# Autodesk Inventor assembly: saddle cart
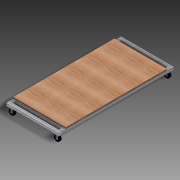
[picture p0: Inventor's stored thumbnail of the model, 180x180]
Saved by Autodesk Inventor 2013 (Build 170138000, 138)
## iProperties
Created: 2013-01-03
Part Number: saddle cart
Document SubType Name: Assembly
Designer: Arpan
Author: Arpan
## Documents named in this file (7)
- C:\Users\Arpan\Documents\Robotics 2013\Cart- Take 2\saddle cart.iam
- C:\Users\Arpan\Documents\Robotics 2013\Cart- Take 2\56 piece.ipt
- C:\Users\Arpan\Documents\Robotics 2013\Cart- Take 2\28 piece.ipt
- C:\Users\Arpan\Documents\Robotics 2013\Cart- Take 2\25 piece.ipt
- C:\Users\Arpan\Documents\Robotics 2013\Cart- Take 2\2.5 piece.ipt
- C:\Users\Arpan\Documents\Robotics 2013\Cart- Take 2\saddle cart top.ipt
- C:\Users\Arpan\Documents\Robotics 2013\Cart- Take 2\small caster\small caster.iam
## Components (15 placed, 6 different names)
1. 56 piece:1 — Mate:1, Flush:1, Flush:2, Mate:4, Flush:7, Mate:5, Flush:8, Mate:14, Mate:15, Flush:14, Flush:18, Flush:22
2. 56 piece:2 — Flush:3, Flush:4, Mate:2, Mate:3, Flush:5, Flush:6, Mate:12, Mate:13, Flush:15, Mate:19, Flush:20
3. 28 piece:1 — Mate:1, Flush:1, Flush:2, Flush:3, Flush:4, Mate:2, Mate:17, Flush:16, Mate:18, Flush:17
4. 28 piece:2 — Mate:3, Flush:5, Flush:6, Mate:7, Flush:19, Mate:20, Flush:21
5. 25 piece:1 — Mate:4, Flush:7, Mate:6, Mate:7, Flush:11, Mate:10, Flush:12, Mate:11, Mate:16
6. 25 piece:2 — Mate:5, Flush:8, Mate:6, Mate:8, Flush:9, Flush:10, Mate:9, Flush:13
7. 2.5 piece:1 — Mate:8, Flush:9, Mate:13
8. 2.5 piece:2 — Flush:10, Mate:9, Mate:14
9. 2.5 piece:3 — Flush:11, Mate:10, Mate:15
10. 2.5 piece:4 — Flush:12, Mate:11, Mate:12
11. saddle cart top:1 — Mate:16, Flush:13, Flush:14
12. small caster:1 [sub-assembly] — Mate:19, Flush:19, Flush:20
13. small caster:2 [sub-assembly] — Mate:17, Flush:15, Flush:16
14. small caster:3 [sub-assembly] — Mate:18, Flush:17, Flush:18
15. small caster:4 [sub-assembly] — Mate:20, Flush:21, Flush:22
## Relationships (42: Flush 22, Mate 20)
- Mate:1: 56 piece:1 ↔ 28 piece:1
- Flush:1: 56 piece:1 ↔ 28 piece:1
- Flush:2: 56 piece:1 ↔ 28 piece:1
- Flush:3: 56 piece:2 ↔ 28 piece:1
- Flush:4: 56 piece:2 ↔ 28 piece:1
- Mate:2: 56 piece:2 ↔ 28 piece:1
- Mate:3: 56 piece:2 ↔ 28 piece:2
- Flush:5: 56 piece:2 ↔ 28 piece:2
- Flush:6: 56 piece:2 ↔ 28 piece:2
- Mate:4: 56 piece:1 ↔ 25 piece:1
- Flush:7: 56 piece:1 ↔ 25 piece:1
- Mate:5: 56 piece:1 ↔ 25 piece:2
- Flush:8: 56 piece:1 ↔ 25 piece:2
- Mate:6 (1244.6 mm): 25 piece:1 ↔ 25 piece:2
- Mate:7 (50.8 mm): 28 piece:2 ↔ 25 piece:1
- Mate:8: 25 piece:2 ↔ 2.5 piece:1
- Flush:9: 25 piece:2 ↔ 2.5 piece:1
- Flush:10: 25 piece:2 ↔ 2.5 piece:2
- Mate:9: 25 piece:2 ↔ 2.5 piece:2
- Flush:11: 25 piece:1 ↔ 2.5 piece:3
- Mate:10: 25 piece:1 ↔ 2.5 piece:3
- Flush:12: 25 piece:1 ↔ 2.5 piece:4
- Mate:11: 25 piece:1 ↔ 2.5 piece:4
- Mate:12 (3.175 mm): 56 piece:2 ↔ 2.5 piece:4
- Mate:13 (3.175 mm): 56 piece:2 ↔ 2.5 piece:1
- Mate:14 (3.175 mm): 56 piece:1 ↔ 2.5 piece:2
- Mate:15 (3.175 mm): 56 piece:1 ↔ 2.5 piece:3
- Mate:16: 25 piece:1 ↔ saddle cart top:1
- Flush:13: 25 piece:2 ↔ saddle cart top:1
- Flush:14: 56 piece:1 ↔ saddle cart top:1
- Mate:17: 28 piece:1 ↔ small caster:2
- Flush:15: 56 piece:2 ↔ small caster:2
- Flush:16: 28 piece:1 ↔ small caster:2
- Mate:18: 28 piece:1 ↔ small caster:3
- Flush:17: 28 piece:1 ↔ small caster:3
- Flush:18: 56 piece:1 ↔ small caster:3
- Mate:19: 56 piece:2 ↔ small caster:1
- Flush:19: 28 piece:2 ↔ small caster:1
- Flush:20: 56 piece:2 ↔ small caster:1
- Mate:20: 28 piece:2 ↔ small caster:4
- Flush:21: 28 piece:2 ↔ small caster:4
- Flush:22: 56 piece:1 ↔ small caster:4
